# Autodesk Inventor assembly: Assem1
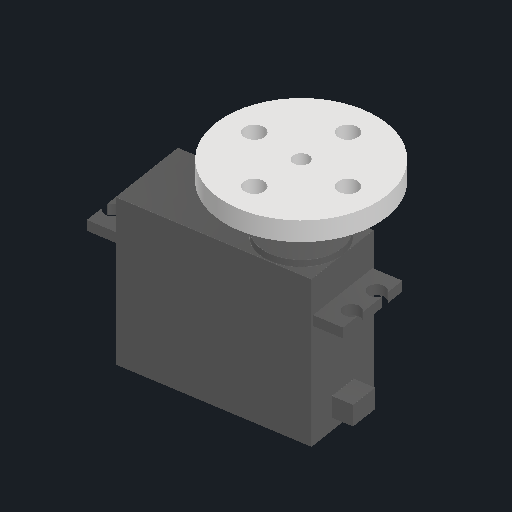
[picture p0: Inventor's stored thumbnail of the model, 512x512]
Saved by Autodesk Inventor 2027.1 (Build 311270010, 270A)
## iProperties
Created: 2021-09-09
Part Number: Assem1
Document SubType Name: Assembly
Designer: daniel
Sending System: SOLIDWORKS 2020
Last Saved Date: 2021-09-09
last saved by: DIMA
Author: daniel
## Documents named in this file (4)
- E:\Apps\AutodeskInventor\University\MCT333_Design_of_Mechatronics_Systems_1\CAD\off_the_shelf_components\standard-servo-motor-black-1.snapshot.7\Assem1\Assem1.iam
- E:\Apps\AutodeskInventor\University\MCT333_Design_of_Mechatronics_Systems_1\CAD\off_the_shelf_components\standard-servo-motor-black-1.snapshot.7\Assem1\body.ipt
- E:\Apps\AutodeskInventor\University\MCT333_Design_of_Mechatronics_Systems_1\CAD\FEED and Sorting\Part25.ipt
- E:\Apps\AutodeskInventor\University\MCT333_Design_of_Mechatronics_Systems_1\CAD\FEED and Sorting\Part57.ipt
## Components (3 placed, 3 different names)
1. body-1 — Mate:1, Mate:2
2. Part25:1 — Mate:3, Mate:4, Mate:5
3. Part57:2 — Mate:1, Mate:2, Mate:3, Mate:4, Mate:5
## Relationships (5: Mate 5)
- Mate:1: body-1 ↔ Part57:2
- Mate:2: body-1 ↔ Part57:2
- Mate:3: Part25:1 ↔ Part57:2
- Mate:4: Part25:1 ↔ Part57:2
- Mate:5: Part25:1 ↔ Part57:2
